# Autodesk Inventor assembly: throwing_mechanism
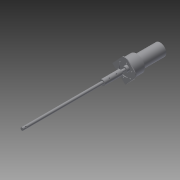
[picture p0: Inventor's stored thumbnail of the model, 180x180]
Saved by Autodesk Inventor 2015 (Build 190159000, 159)
## iProperties
Created: 2017-09-26
Part Number: throwing_mechanism
Document SubType Name: Assembly
Designer: Anshul
Author: Anshul
## Documents named in this file (5)
- E:\robocon\throwing bot\throwing_mechanism.iam
- E:\robocon\throwing bot\metal_shaft.ipt
- E:\robocon\throwing bot\offcenter_L_clamp.ipt
- E:\robocon\throwing bot\offcentered_shaft_dc_and_encoder.ipt
- E:\robocon\throwing bot\shaft_to_dc_coupler.ipt
## Components (4 placed, 4 different names)
1. metal_shaft:1 — Mate:6, Mate:7
2. offcenter_L_clamp:1 — Mate:3, Mate:4, Mate:5
3. offcentered_shaft_dc_and_encoder:1 — Mate:1, Mate:2, Mate:3, Mate:4, Mate:5
4. shaft_to_dc_coupler:1 — Mate:1, Mate:2, Mate:6, Mate:7
## Relationships (7: Mate 7)
- Mate:1: offcentered_shaft_dc_and_encoder:1 ↔ shaft_to_dc_coupler:1
- Mate:2: offcentered_shaft_dc_and_encoder:1 ↔ shaft_to_dc_coupler:1
- Mate:3: offcenter_L_clamp:1 ↔ offcentered_shaft_dc_and_encoder:1
- Mate:4: offcenter_L_clamp:1 ↔ offcentered_shaft_dc_and_encoder:1
- Mate:5: offcenter_L_clamp:1 ↔ offcentered_shaft_dc_and_encoder:1
- Mate:6: metal_shaft:1 ↔ shaft_to_dc_coupler:1
- Mate:7: metal_shaft:1 ↔ shaft_to_dc_coupler:1
